# Autodesk Inventor assembly: TapeMeasureAssemblyVersion1
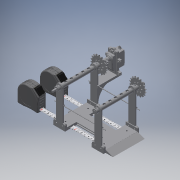
[picture p0: Inventor's stored thumbnail of the model, 180x180]
Saved by Autodesk Inventor 2019 (Build 230136000, 136)
## iProperties
Created: 2018-11-08
Part Number: TapeMeasureAssemblyVersion1
Document SubType Name: Assembly
Designer: Ashley
Author: Ashley
## Documents named in this file (17)
- C:\Users\mrhftc\repositories\design\inventor\2018-2019\Tape Measure Braket\Version One\Tape Measure Bracket Assembly V1.iam
- C:\Users\mrhftc\repositories\design\inventor\2018-2019\Tape Measure Braket\Version One\Bracket Bottom V1.ipt
- C:\Users\mrhftc\repositories\design\inventor\2018-2019\Tape Measure Braket\Tape Measure\Tape Measure Edited.iam
- C:\Users\mrhftc\repositories\design\inventor\2018-2019\Tape Measure Braket\Version One\Bracket Top V1.ipt
- C:\Users\mrhftc\repositories\design\inventor\2018-2019\Tape Measure Braket\Version One\Side V1.ipt
- C:\Users\mrhftc\repositories\design\inventor\Imported Components\goBilda\Bearing6mmID.ipt
- C:\Users\mrhftc\repositories\design\inventor\2018-2019\Tape Measure Braket\Finished Parts\Spinner94mmDShaft.ipt
- C:\Users\mrhftc\repositories\design\inventor\Imported Components\goBilda\DShaft140mm.ipt
- C:\Users\mrhftc\repositories\design\inventor\Imported Components\goBilda\Collar6mm\SetScrewCollar6mmboreassembly.iam
- C:\Users\mrhftc\repositories\design\inventor\Imported Components\goBilda\DShaft160mm.ipt
- C:\Users\mrhftc\repositories\design\inventor\2018-2019\Tape Measure Braket\Finished Parts\2mmAxel.ipt
- C:\Users\mrhftc\repositories\design\inventor\Imported Components\goBilda\CampingHub\ClampingHub assembly.iam
- C:\Users\mrhftc\repositories\design\inventor\Imported Components\goBilda\8mmPlasticPitchSproket.ipt
- C:\Users\mrhftc\repositories\design\inventor\Imported Components\goBilda\Servo To Shaft\ServoToShaftCoupler.iam
- C:\Users\mrhftc\repositories\design\inventor\Imported Components\goBilda\goBildaServo.ipt
- C:\Users\mrhftc\repositories\design\inventor\Imported Components\goBilda\1802SeriesServoFrame.ipt
- C:\Users\mrhftc\repositories\design\inventor\2018-2019\Tape Measure Braket\Version One\Side Servo V1.ipt
## Components (29 placed, 29 different names)
1. Bracket Bottom — Mate:1
2. Tape Measure Right [sub-assembly]
3. Tape Measure Left [sub-assembly]
4. Bracket Top
5. Back Right Side
6. Front Right Side — Mate:1, Insert:2, Insert:11
7. Front Left Side — Insert:3, Insert:10
8. Back Right Bearing — Insert:17
9. Front Right Bearing — Insert:2
10. Front Left Beaing — Insert:3
11. Front Left BEaring — Insert:23
12. Back Spinner — Insert:22
13. Front Spinner — Insert:6
14. Front Right Collar [sub-assembly]
15. Front Axel — Insert:6, Insert:8, Insert:14
16. Front Left Collar [sub-assembly] — Insert:8
17. Back Left Collar [sub-assembly]
18. Back Right Collar [sub-assembly] — Insert:18
19. Back Axel — Insert:17, Insert:18, Insert:19, Insert:20, Insert:22
20. Left axel — Insert:10
21. Right Axel — Insert:11
22. Front Sproket — Insert:12
23. Front Claming Hub [sub-assembly] — Insert:12, Insert:14
24. Back Sproket
25. Back Clamping Hub [sub-assembly] — Insert:19
26. Servo To Shaft Coupler [sub-assembly] — Insert:20, Insert:21
27. Servo — Insert:21, Mate:3
28. Servo Frame — Mate:3
29. Side Servo V1:1 — Insert:23
## Relationships (18: Insert 16, Mate 2)
- Mate:1: Bracket Bottom ↔ Front Right Side
- Insert:2: Front Right Side ↔ Front Right Bearing
- Insert:3: Front Left Side ↔ Front Left Beaing
- Insert:6 (17 mm): Front Spinner ↔ Front Axel
- Insert:8 (14 mm): Front Axel ↔ Front Left Collar
- Insert:10 (-30 mm): Front Left Side ↔ Left axel
- Insert:11 (-30 mm): Front Right Side ↔ Right Axel
- Insert:12 (-1 mm): Front Sproket ↔ Front Claming Hub
- [Insert] (-1 mm): Back Sproket ↔ Back Clamping Hub
- Insert:14 (1 mm): Front Axel ↔ Front Claming Hub
- Insert:17 (20 mm): Back Right Bearing ↔ Back Axel
- Insert:18 (12 mm): Back Right Collar ↔ Back Axel
- Insert:19 (11 mm): Back Axel ↔ Back Clamping Hub
- Insert:20 (-6 mm): Back Axel ↔ Servo To Shaft Coupler
- Insert:21 (-3 mm): Servo To Shaft Coupler ↔ Servo
- Mate:3: Servo ↔ Servo Frame
- Insert:22 (40 mm): Back Spinner ↔ Back Axel
- Insert:23: Front Left BEaring ↔ Side Servo V1:1
## Named parameters: d26_d25 = -1 mm
